# Autodesk Inventor assembly: Motors with Screws
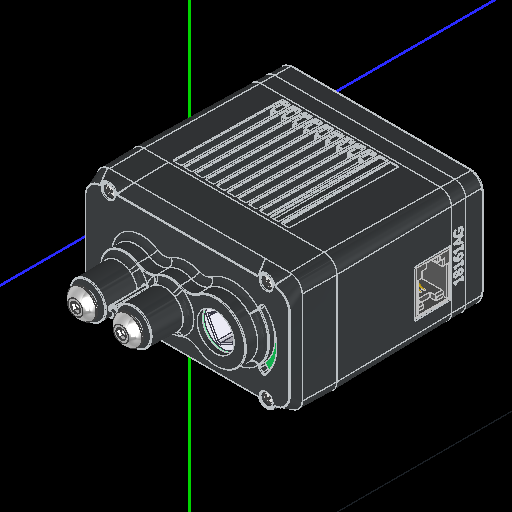
[picture p0: Inventor's stored thumbnail of the model, 512x512]
Saved by Autodesk Inventor 2025.2 (Build 292293000, 293)
## iProperties
Created: 2022-08-18
Part Number: Motors with Screws
Document SubType Name: Assembly
Designer: ylu12
Author: ylu12
## Documents named in this file (5)
- C:\Users\cloudy\Documents\Inventor\AURA\!VEX-CAD-Inventor\Electronics\Motors with Screws\SteelM-HexS.iam
- C:\Users\cloudy\Documents\Inventor\AURA\!VEX-CAD-Inventor\Electronics\V5 Motor.ipt
- C:\Users\cloudy\Documents\Inventor\AURA\!VEX-CAD-Inventor\Structure\Hardware\Screw Steel - Hex\SScrew Hex Smooth .500.ipt
- C:\Users\ylu12\Documents\GitHub\VEX-CAD-Inventor\Structure\Hardware\Screw Steel - Hex.ipt
- C:\Users\cloudy\Documents\Inventor\AURA\!VEX-CAD-Inventor\Electronics\Motors with Screws.iam
## Components (3 placed, 2 different names)
1. V5 Motor:1 — Insert:1, Insert:2
2. SScrew Hex Smooth .500:1 — Insert:1
3. SScrew Hex Smooth .500:2 — Insert:2
## Relationships (2: Insert 2)
- Insert:1 (1.1906 mm): V5 Motor:1 ↔ SScrew Hex Smooth .500:1
- Insert:2 (1.1906 mm): V5 Motor:1 ↔ SScrew Hex Smooth .500:2
## Named parameters: Thickness = 1.19063 mm
